# Autodesk Inventor assembly: ToASI-6
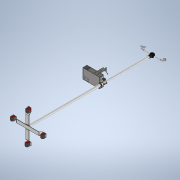
[picture p0: Inventor's stored thumbnail of the model, 180x180]
Saved by Autodesk Inventor 2020.3 (Build 243373000, 373)
## iProperties
Created: 2020-08-01
Part Number: ToASI-6
Document SubType Name: Assembly
Designer: Bruno
Author: Bruno
## Documents named in this file (10)
- C:\Users\Bruno\Desktop\Github\CAD\Inventor\For ASI\ToASI-6.iam
- C:\Users\Bruno\Desktop\Github\CAD\Inventor\For ASI\ToASI-4.iam
- C:\Users\Bruno\Desktop\Github\CAD\Inventor\Heater-Box\Glass vase _ flow meter fixer\Glass fixer plate.ipt
- C:\Users\Bruno\Desktop\Github\CAD\Inventor\Heater-Box\Glass vase _ flow meter fixer\DIN912 M4x0.7x10-8.8 socket head screw.ipt
- C:\Users\Bruno\Desktop\Github\CAD\Inventor\Heater-Box\IV stand fixer\Box-iv stand Connector.ipt
- C:\Users\Bruno\Desktop\Github\CAD\Inventor\Heater-Box\IV stand fixer\DIN912 M4x0.7x10-8.8 socket head screw.ipt
- C:\Users\Bruno\Desktop\Github\CAD\Inventor\Heater-Box\IV stand fixer\Split Washer DIN127B D4.ipt
- C:\Users\Bruno\Desktop\Github\CAD\Inventor\Heater-Box\IV stand fixer\DIN934-M4 nut.ipt
- C:\Users\Bruno\Desktop\Github\CAD\Inventor\Heater-Box\IV stand fixer\Star Knob 1-4UNC.ipt
- C:\Users\Bruno\Desktop\Github\CAD\Inventor\Auxiliary Components\IV Stand.ipt
## Components (18 placed, 8 different names)
1. ToASI-4:1 [sub-assembly] — Cylindrical:1, Cylindrical:4, Cylindrical:5
2. Glass fixer plate:1 — Cylindrical:1, Cylindrical:2, Cylindrical:3
3. DIN912 M4x0.7x10-8.8 socket head screw:1 — Cylindrical:3
4. DIN912 M4x0.7x10-8.8 socket head screw:2 — Cylindrical:2
5. Box-iv stand Connector:1 — Cylindrical:4, Cylindrical:6, Cylindrical:7, Cylindrical:14, Cylindrical:15, Cylindrical:16
6. Box-iv stand Connector:2 — Cylindrical:5, Cylindrical:8, Cylindrical:9, Cylindrical:10, Cylindrical:11, Cylindrical:17
7. DIN912 M4x0.7x10-8.8 socket head screw:3 — Cylindrical:7
8. DIN912 M4x0.7x10-8.8 socket head screw:4 — Cylindrical:9
9. DIN912 M4x0.7x10-8.8 socket head screw:5 — Cylindrical:6
10. DIN912 M4x0.7x10-8.8 socket head screw:6 — Cylindrical:8
11. DIN912 M4x0.7x10-8.8 socket head screw:7 — Cylindrical:12
12. DIN912 M4x0.7x10-8.8 socket head screw:8 — Cylindrical:13
13. Split Washer DIN127B D4:1 — Cylindrical:10, Cylindrical:12
14. Split Washer DIN127B D4:2 — Cylindrical:11, Cylindrical:13
15. DIN934-M4 nut:1 — Cylindrical:15
16. DIN934-M4 nut:2 — Cylindrical:14
17. Star Knob 1-4UNC:1 — Cylindrical:16
18. IV Stand:1 — Cylindrical:17
## Relationships (17: CylindricalJoint 17)
- Cylindrical:1: ToASI-4:1 ↔ Glass fixer plate:1
- Cylindrical:2: Glass fixer plate:1 ↔ DIN912 M4x0.7x10-8.8 socket head screw:2
- Cylindrical:3: Glass fixer plate:1 ↔ DIN912 M4x0.7x10-8.8 socket head screw:1
- Cylindrical:4: ToASI-4:1 ↔ Box-iv stand Connector:1
- Cylindrical:5: ToASI-4:1 ↔ Box-iv stand Connector:2
- Cylindrical:6: Box-iv stand Connector:1 ↔ DIN912 M4x0.7x10-8.8 socket head screw:5
- Cylindrical:7: Box-iv stand Connector:1 ↔ DIN912 M4x0.7x10-8.8 socket head screw:3
- Cylindrical:8: Box-iv stand Connector:2 ↔ DIN912 M4x0.7x10-8.8 socket head screw:6
- Cylindrical:9: Box-iv stand Connector:2 ↔ DIN912 M4x0.7x10-8.8 socket head screw:4
- Cylindrical:10: Box-iv stand Connector:2 ↔ Split Washer DIN127B D4:1
- Cylindrical:11: Box-iv stand Connector:2 ↔ Split Washer DIN127B D4:2
- Cylindrical:12: DIN912 M4x0.7x10-8.8 socket head screw:7 ↔ Split Washer DIN127B D4:1
- Cylindrical:13: DIN912 M4x0.7x10-8.8 socket head screw:8 ↔ Split Washer DIN127B D4:2
- Cylindrical:14: Box-iv stand Connector:1 ↔ DIN934-M4 nut:2
- Cylindrical:15: Box-iv stand Connector:1 ↔ DIN934-M4 nut:1
- Cylindrical:16: Box-iv stand Connector:1 ↔ Star Knob 1-4UNC:1
- Cylindrical:17: Box-iv stand Connector:2 ↔ IV Stand:1
